# Autodesk Inventor assembly: N20Module_MIR
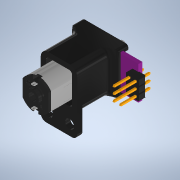
[picture p0: Inventor's stored thumbnail of the model, 180x180]
Saved by Autodesk Inventor 2022 (Build 260153000, 153)
## iProperties
Created: 2021-12-07
Part Number: N20Module_MIR
Document SubType Name: Assembly
Designer: JK
Author: JK
## Documents named in this file (6)
- C:\Users\JK\Documents\Inventor\N20 Leg Actuator\N20-Leg-Actuator\CADfiles\N20Module\N20Module_MIR.iam
- C:\Users\JK\Documents\Inventor\N20 Leg Actuator\N20-Leg-Actuator\CADfiles\N20Module\Brushed DC Motor v8_MIR.iam
- C:\Users\JK\Documents\Inventor\N20 Leg Actuator\N20-Leg-Actuator\CADfiles\N20Module\MotorCase_MIR.ipt
- C:\Users\JK\Documents\Inventor\N20 Leg Actuator\N20-Leg-Actuator\CADfiles\N20Module\adapter.ipt
- C:\Users\JK\Documents\Inventor\N20 Leg Actuator\N20-Leg-Actuator\CADfiles\N20Module\AngleSensor.ipt
- C:\Users\JK\Documents\Inventor\N20 Leg Actuator\N20-Leg-Actuator\CADfiles\N20Module\2x3pinheader.iam
## Components (5 placed, 5 different names)
1. Brushed DC Motor v8_MIR:1 [sub-assembly] — Nivelación:1, Coincidencia:2, Coincidencia:1, Coincidencia:5, Ángulo:2, Coincidencia:6
2. MotorCase_MIR:1 — Nivelación:1, Coincidencia:2, Coincidencia:1, Coincidencia:7, Ángulo:3
3. adapter:1 — Coincidencia:5, Ángulo:2
4. AngleSensor:1 — Coincidencia:6, Coincidencia:7, Ángulo:3, Coincidencia:8, Nivelación:2, Nivelación:3
5. 2x3pinheader:1 [sub-assembly] — Coincidencia:8, Nivelación:2, Nivelación:3
## Relationships (11: Mate 6, Flush 3, Angle 2)
- Nivelación:1 [Flush]: Brushed DC Motor v8_MIR:1 ↔ MotorCase_MIR:1
- Coincidencia:2 [Mate] (0.15 mm): Brushed DC Motor v8_MIR:1 ↔ MotorCase_MIR:1
- Coincidencia:1 [Mate] (0.15 mm): Brushed DC Motor v8_MIR:1 ↔ MotorCase_MIR:1
- Coincidencia:5 [Mate]: Brushed DC Motor v8_MIR:1 ↔ adapter:1
- Ángulo:2 [Angle] (0 deg): Brushed DC Motor v8_MIR:1 ↔ adapter:1
- Coincidencia:6 [Mate]: Brushed DC Motor v8_MIR:1 ↔ AngleSensor:1
- Coincidencia:7 [Mate]: MotorCase_MIR:1 ↔ AngleSensor:1
- Ángulo:3 [Angle] (0 deg): MotorCase_MIR:1 ↔ AngleSensor:1
- Coincidencia:8 [Mate]: AngleSensor:1 ↔ 2x3pinheader:1
- Nivelación:2 [Flush] (-2.54 mm): AngleSensor:1 ↔ 2x3pinheader:1
- Nivelación:3 [Flush] (2.7 mm): AngleSensor:1 ↔ 2x3pinheader:1
